# Autodesk Inventor assembly: Full Truck
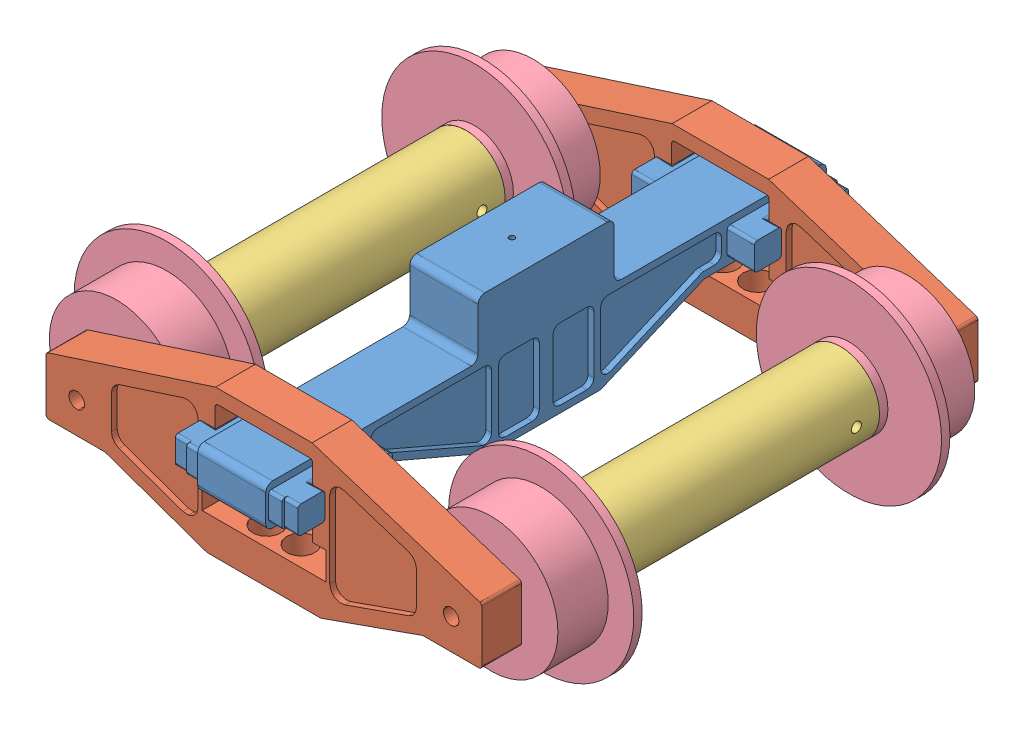
[picture p0: shaded view drawn from the shape stored in the file]
Saved by Autodesk Inventor 2023 (Build 270158030, 158C)
## iProperties
Created: 2023-02-14
Part Number: Full Truck
Document SubType Name: Assembly
Designer: jeremyy
Author: jeremyy
## Documents named in this file (4)
- \\andrew.ad.cmu.edu\users\users1\jeremyy\Documents\Inventor\CMU Bridge\Car\Full Truck.iam
- \\andrew.ad.cmu.edu\users\users1\jeremyy\Documents\Inventor\CMU Bridge\Car\Car_truck.ipt
- \\andrew.ad.cmu.edu\users\users1\jeremyy\Documents\Inventor\CMU Bridge\Wheel.ipt
- \\andrew.ad.cmu.edu\users\users1\jeremyy\Documents\Inventor\CMU Bridge\Car\Wheel_axis.ipt
## Components (7 placed, 3 different names)
1. Car_truck:1 — Tangent:1, Mate:1, Tangent:2, Mate:2, Tangent:3, Mate:3, Tangent:4, Mate:4
2. Wheel:1 — Tangent:1, Mate:1
3. Wheel:2 — Tangent:2, Mate:2, Tangent:5
4. Wheel:3 — Tangent:3, Mate:3, Tangent:6, Mate:6, Mate:7
5. Wheel:4 — Tangent:4, Mate:4, Mate:5
6. Wheel_axis:1 — Tangent:5, Mate:5
7. Wheel_axis:2 — Tangent:6, Mate:6, Mate:7
## Relationships (13: Mate 7, Tangent 6)
- Tangent:1: Car_truck:1 ↔ Wheel:1
- Mate:1: Car_truck:1 ↔ Wheel:1
- Tangent:2: Car_truck:1 ↔ Wheel:2
- Mate:2: Car_truck:1 ↔ Wheel:2
- Tangent:3: Car_truck:1 ↔ Wheel:3
- Mate:3: Car_truck:1 ↔ Wheel:3
- Tangent:4: Car_truck:1 ↔ Wheel:4
- Mate:4: Car_truck:1 ↔ Wheel:4
- Tangent:5: Wheel:2 ↔ Wheel_axis:1
- Mate:5: Wheel:4 ↔ Wheel_axis:1
- Tangent:6: Wheel:3 ↔ Wheel_axis:2
- Mate:6: Wheel:3 ↔ Wheel_axis:2
- Mate:7: Wheel:3 ↔ Wheel_axis:2
